# Autodesk Inventor assembly: Lower_Arm_v3_Assembly
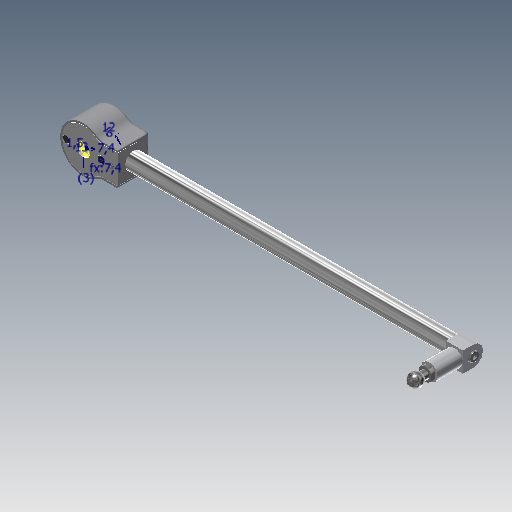
[picture p0: Inventor's stored thumbnail of the model, 512x512]
Saved by Autodesk Inventor 2021.4 (Build 254397000, 397)
## iProperties
Created: 2022-07-05
Part Number: Lower_Arm_v3_Assembly
Material: Generisch
Document SubType Name: Assembly
Designer: alexw
Mass: 38.9031 g
Surface Area: 225.46 cm^2
Volume: 16.1811 cm^3
Density: 2.40423 g/cm^3
Distance2ShaftCenter: 4,000 mm
Author: alexw
## Documents named in this file (9)
- C:\Users\alexw\Documents\Inventor\Projects\03_CurrentProjects\MasterThesis\TrainingConsol_220422\Workgroups\Workgroup\Lower_Arm_v3_Assembly.iam
- C:\Users\alexw\Documents\Inventor\Projects\03_CurrentProjects\MasterThesis\TrainingConsol_220422\Workgroups\Workgroup\Lower_Arm_Shaft.ipt
- C:\Users\alexw\Documents\Inventor\Projects\03_CurrentProjects\MasterThesis\TrainingConsol_220422\Workgroups\Workgroup\Ball_Joint_Ball.ipt
- C:\Users\alexw\Documents\Inventor\Projects\03_CurrentProjects\MasterThesis\TrainingConsol_220422\Workgroups\Workgroup\LowerArm_Cover.ipt
- C:\Users\alexw\Documents\Inventor\Projects\03_CurrentProjects\MasterThesis\TrainingConsol_220422\Workgroups\Workgroup\ContentCenter\en-US\ISO 7046-1 H(1)\ISO 7046-1 - M2 x 10_ - 4.8 - H - ISO.ipt
- C:\Users\alexw\Documents\Inventor\Projects\03_CurrentProjects\MasterThesis\TrainingConsol_220422\Workgroups\Workgroup\LowerArm_JointConnector_Prox_v2_printversion.ipt
- C:\Users\alexw\Documents\Inventor\Projects\03_CurrentProjects\MasterThesis\TrainingConsol_220422\Workgroups\Workgroup\Endeffector_Fixationl.ipt
- C:\Users\alexw\Documents\Inventor\Projects\03_CurrentProjects\MasterThesis\TrainingConsol_220422\Workgroups\Workgroup\ContentCenter\en-US\ISO 4762(2)\ISO 4762 - M3 x 16ISO.ipt
- C:\Users\alexw\Documents\Inventor\Projects\03_CurrentProjects\MasterThesis\TrainingConsol_220422\Workgroups\Workgroup\Downloads\din_913-m3x5-45h.ipt
## Components (9 placed, 8 different names)
1. Lower_Arm_Shaft:1 — Mate:26, Mate:38, Flush:3, Mate:42, Mate:43, Tangent:1
2. Ball_Joint_Ball:1 — Mate:44, Mate:45, Angle:2
3. LowerArm_JointConnector_Prox_v2_printversion:1 — Flush:2, Mate:32, Mate:35, Mate:38, Flush:3, Flush:4, Flush:5, Mate:39, Mate:40, Mate:41, Angle:1, Mate:48
4. LowerArm_Cover:1 — Flush:2, Mate:40, Mate:41
5. ISO 7046-1 H M2 x 10 - 4.8 - H:1 — Mate:32
6. ISO 7046-1 H M2 x 10 - 4.8 - H:4 — Mate:35
7. Endeffector_Fixationl:1 — Mate:42, Angle:1, Mate:43, Mate:44, Mate:45, Angle:2, Mate:46, Mate:47
8. ISO 4762 M3 x 16:1 — Mate:46, Mate:47
9. din_913-m3x5-45h:1 — Mate:48, Tangent:1
## Relationships (21: Mate 14, Flush 4, Angle 2, Tangent 1)
- Mate:26: Lower_Arm_Shaft:1
- Flush:2: LowerArm_JointConnector_Prox_v2_printversion:1 ↔ LowerArm_Cover:1
- Mate:32: LowerArm_JointConnector_Prox_v2_printversion:1 ↔ ISO 7046-1 H M2 x 10 - 4.8 - H:1
- Mate:35: LowerArm_JointConnector_Prox_v2_printversion:1 ↔ ISO 7046-1 H M2 x 10 - 4.8 - H:4
- Mate:38: Lower_Arm_Shaft:1 ↔ LowerArm_JointConnector_Prox_v2_printversion:1
- Flush:3: Lower_Arm_Shaft:1 ↔ LowerArm_JointConnector_Prox_v2_printversion:1
- Flush:4: LowerArm_JointConnector_Prox_v2_printversion:1
- Flush:5: LowerArm_JointConnector_Prox_v2_printversion:1
- Mate:39: LowerArm_JointConnector_Prox_v2_printversion:1
- Mate:40: LowerArm_JointConnector_Prox_v2_printversion:1 ↔ LowerArm_Cover:1
- Mate:41: LowerArm_JointConnector_Prox_v2_printversion:1 ↔ LowerArm_Cover:1
- Mate:42: Lower_Arm_Shaft:1 ↔ Endeffector_Fixationl:1
- Angle:1 (0 deg): LowerArm_JointConnector_Prox_v2_printversion:1 ↔ Endeffector_Fixationl:1
- Mate:43: Lower_Arm_Shaft:1 ↔ Endeffector_Fixationl:1
- Mate:44: Ball_Joint_Ball:1 ↔ Endeffector_Fixationl:1
- Mate:45: Ball_Joint_Ball:1 ↔ Endeffector_Fixationl:1
- Angle:2 (0 deg): Ball_Joint_Ball:1 ↔ Endeffector_Fixationl:1
- Mate:46: Endeffector_Fixationl:1 ↔ ISO 4762 M3 x 16:1
- Mate:47: Endeffector_Fixationl:1 ↔ ISO 4762 M3 x 16:1
- Mate:48: LowerArm_JointConnector_Prox_v2_printversion:1 ↔ din_913-m3x5-45h:1
- Tangent:1: Lower_Arm_Shaft:1 ↔ din_913-m3x5-45h:1
## Named parameters: Distance2ShaftCenter = 4 mm
